# Autodesk Inventor assembly: UpperBody
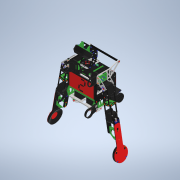
[picture p0: Inventor's stored thumbnail of the model, 180x180]
Saved by Autodesk Inventor 2020 (Build 240168000, 168)
## iProperties
Created: 2022-01-14
Part Number: UpperBody
Document SubType Name: Assembly
Designer: Masato Kubotera
Mass: 1918.95 g
Surface Area: 7006.93 cm^2
Volume: 1229.13 cm^3
Density: 1.56122 g/cm^3
Author: Masato Kubotera
## Documents named in this file (8)
- C:\Users\MasatoKubotera\Documents\Inventor\SUSTAINA-OP\UpperBody\UpperBody.iam
- C:\Users\MasatoKubotera\Documents\Inventor\SUSTAINA-OP\UpperBody\Trunk\Trunk.iam
- C:\Users\MasatoKubotera\Documents\Inventor\SUSTAINA-OP\UpperBody\Head\Head.iam
- C:\Users\MasatoKubotera\Documents\Inventor\SUSTAINA-OP\UpperBody\Arm\Shoulder.iam
- C:\Users\MasatoKubotera\Documents\Inventor\SUSTAINA-OP\UpperBody\Arm\UpperArm.iam
- C:\Users\MasatoKubotera\Documents\Inventor\SUSTAINA-OP\UpperBody\Arm\ForeArm.iam
- C:\Users\MasatoKubotera\Documents\Inventor\SUSTAINA-OP\UpperBody\Arm\UpperArm_MIR.iam
- C:\Users\MasatoKubotera\Documents\Inventor\SUSTAINA-OP\UpperBody\Cockpit\Cockpit.iam
## Components (9 placed, 7 different names)
1. Trunk:1 [sub-assembly] — フラッシュ:1, フラッシュ:2, フラッシュ:3, 挿入:1, 角度:1, 挿入:2, 挿入:3, 角度:2, 角度:3, 挿入:11
2. Head:1 [sub-assembly] — 挿入:1, 角度:1
3. Shoulder:1 [sub-assembly] — 挿入:2, 角度:2, 挿入:4, 角度:4
4. Shoulder:2 [sub-assembly] — 挿入:3, 角度:3, 挿入:9, 角度:7
5. UpperArm:1 [sub-assembly] — 挿入:4, 角度:4, 挿入:6, 角度:6
6. ForeArm:1 [sub-assembly] — 挿入:6, 角度:6
7. ForeArm:2 [sub-assembly] — 挿入:10, 角度:8
8. UpperArm_MIR:1 [sub-assembly] — 挿入:9, 挿入:10, 角度:7, 角度:8
9. Cockpit:1 [sub-assembly] — 挿入:11, 角度:9
## Relationships (19: Insert 8, Angle 8, Flush 3)
- フラッシュ:1 [Flush]: Trunk:1
- フラッシュ:2 [Flush]: Trunk:1
- フラッシュ:3 [Flush]: Trunk:1
- 挿入:1 [Insert]: Trunk:1 ↔ Head:1
- 角度:1 [Angle] (0 deg): Trunk:1 ↔ Head:1
- 挿入:2 [Insert]: Trunk:1 ↔ Shoulder:1
- 挿入:3 [Insert]: Trunk:1 ↔ Shoulder:2
- 角度:2 [Angle] (0 deg): Trunk:1 ↔ Shoulder:1
- 角度:3 [Angle] (0 deg): Trunk:1 ↔ Shoulder:2
- 挿入:4 [Insert]: Shoulder:1 ↔ UpperArm:1
- 角度:4 [Angle] (170 deg): Shoulder:1 ↔ UpperArm:1
- 挿入:6 [Insert]: UpperArm:1 ↔ ForeArm:1
- 角度:6 [Angle] (0 deg): UpperArm:1 ↔ ForeArm:1
- 挿入:9 [Insert]: Shoulder:2 ↔ UpperArm_MIR:1
- 挿入:10 [Insert]: ForeArm:2 ↔ UpperArm_MIR:1
- 角度:7 [Angle] (10 deg): Shoulder:2 ↔ UpperArm_MIR:1
- 角度:8 [Angle] (180 deg): ForeArm:2 ↔ UpperArm_MIR:1
- 挿入:11 [Insert] (0.025 mm): Trunk:1 ↔ Cockpit:1
- 角度:9 [Angle] (0 deg): Cockpit:1
